# Autodesk Inventor assembly: CAR_011_VersaPlanetary_v2_Single_Stage_10_1_with_775_Series_Reverse
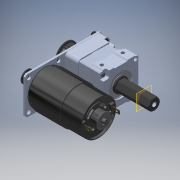
[picture p0: Inventor's stored thumbnail of the model, 180x180]
Saved by Autodesk Inventor 2018 (Build 220112000, 112)
## iProperties
Created: 2016-10-31
Part Number: CAR_011_VersaPlanetary_v2_Single_Stage_10_1_with_775_Series_Reverse
Description: STEP AP214
Document SubType Name: Assembly
Designer: Bobby's PC
Mass: 725.748 g
Surface Area: 818.615 cm^2
Volume: 178.451 cm^3
Density: 4.06694 g/cm^3
Sending System: SolidWorks 2016
Preprocessor: SwSTEP 2.0
Title: 217-4973_1stage_775pro.STEP
Revision Number: ANY
## Documents named in this file (16)
- C:\Users\user\Documents\GrabCAD\New folder\Build season\CAR_011_VersaPlanetary_v2_Single_Stage_10_1_with_775_Series_Reverse.iam
- C:\Users\user\Documents\GrabCAD\New folder\Build season\180 VERSAPLANETARY\217-2625-026 Rev1.ipt
- C:\Users\user\Documents\GrabCAD\New folder\Build season\180 VERSAPLANETARY\217-2742-001 Rev4.ipt
- C:\Users\user\Documents\GrabCAD\New folder\Build season\180 VERSAPLANETARY\217-2625-017 Rev1_9714K61.ipt
- C:\Users\user\Documents\GrabCAD\New folder\Build season\180 VERSAPLANETARY\217-2625-003 Rev1.ipt
- C:\Users\user\Documents\GrabCAD\New folder\Build season\180 VERSAPLANETARY\217-2625-018 Rev1_98541A410.ipt
- C:\Users\user\Documents\GrabCAD\New folder\Build season\180 VERSAPLANETARY\832-1750-Ring-Gear-Screw_SSA0832-0500ZC.ipt
- C:\Users\user\Documents\GrabCAD\New folder\Build season\180 VERSAPLANETARY\217-4649-002 Rev1_SSA0832-0500ZC.ipt
- C:\Users\user\Documents\GrabCAD\New folder\Build season\180 VERSAPLANETARY\217-4347-000 Rev1.ipt
- C:\Users\user\Documents\GrabCAD\New folder\Build season\180 VERSAPLANETARY\217-2820 Rev1_Public.iam
- C:\Users\user\Documents\GrabCAD\New folder\Build season\180 VERSAPLANETARY\217-2816-001 Rev1.ipt
- C:\Users\user\Documents\GrabCAD\New folder\Build season\180 VERSAPLANETARY\217-4649-007 Rev1_94105A824.ipt
- C:\Users\user\Documents\GrabCAD\New folder\Build season\180 VERSAPLANETARY\VersaPlanetary_180_Drive_-_Speed_Reducer.iam
- C:\Users\user\Documents\GrabCAD\New folder\Build season\180 VERSAPLANETARY\VersaPlanetary_180_Drive_Gusset_Kit.ipt
- C:\Users\user\Documents\GrabCAD\New folder\Build season\180 VERSAPLANETARY\12t_x_9mm_Wide_Double_Flange_Aluminum_Pulley_GT2_3mm_RS775_Motor_217-5871.ipt
- C:\Users\user\Documents\GrabCAD\New folder\Build season\180 VERSAPLANETARY\24t_x_9mm_Wide_Double_Flange_Aluminum_Pulley_GT2_3mm_1_2_Hex_Bore_217-5875.ipt
## Components (18 placed, 18 different names)
1. 217-2625-026 Rev1_1
2. 217-2742-001 Rev4_2
3. 217-2742-001 Rev4_3
4. 217-2625-017 Rev1_9714K61_4
5. 217-2625-003 Rev1_5
6. 217-2625-018 Rev1_98541A410_6
7. 832-1750-Ring-Gear-Screw_SSA0832-0500ZC_7 — Insert:10
8. 832-1750-Ring-Gear-Screw_SSA0832-0500ZC_8 — Mate:3, Mate:5
9. 217-4649-002 Rev1_SSA0832-0500ZC_10 — Insert:6
10. 217-4649-002 Rev1_SSA0832-0500ZC_11 — Insert:7, Mate:4
11. 217-4347-000 Rev1_15 — Mate:2, Insert:9, Mate:6
12. 217-2820 Rev1_Public_16 [sub-assembly]
13. 217-2816-001 Rev1_17 — Insert:3
14. 217-4649-007 Rev1_94105A824_19
15. VersaPlanetary_180_Drive_-_Speed_Reducer:1 [sub-assembly] — Insert:3, Insert:4, Insert:8, Mate:3, Mate:4, Mate:5
16. VersaPlanetary_180_Drive_Gusset_Kit:1 — Insert:4, Insert:6, Insert:7, Insert:9, Insert:10
17. 12t_x_9mm_Wide_Double_Flange_Aluminum_Pulley_GT2_3mm_RS775_Motor_217-5871:1 — Mate:2, Flush:2, Mate:6
18. 24t_x_9mm_Wide_Double_Flange_Aluminum_Pulley_GT2_3mm_1_2_Hex_Bore_217-5875:1 — Insert:8, Flush:2
## Relationships (13: Insert 7, Mate 5, Flush 1)
- Insert:3: 217-2816-001 Rev1_17 ↔ VersaPlanetary_180_Drive_-_Speed_Reducer:1
- Insert:4: VersaPlanetary_180_Drive_-_Speed_Reducer:1 ↔ VersaPlanetary_180_Drive_Gusset_Kit:1
- Insert:6 (3.175 mm): 217-4649-002 Rev1_SSA0832-0500ZC_10 ↔ VersaPlanetary_180_Drive_Gusset_Kit:1
- Insert:7: 217-4649-002 Rev1_SSA0832-0500ZC_11 ↔ VersaPlanetary_180_Drive_Gusset_Kit:1
- Insert:8: VersaPlanetary_180_Drive_-_Speed_Reducer:1 ↔ 24t_x_9mm_Wide_Double_Flange_Aluminum_Pulley_GT2_3mm_1_2_Hex_Bore_217-5875:1
- Mate:2: 217-4347-000 Rev1_15 ↔ 12t_x_9mm_Wide_Double_Flange_Aluminum_Pulley_GT2_3mm_RS775_Motor_217-5871:1
- Flush:2: 12t_x_9mm_Wide_Double_Flange_Aluminum_Pulley_GT2_3mm_RS775_Motor_217-5871:1 ↔ 24t_x_9mm_Wide_Double_Flange_Aluminum_Pulley_GT2_3mm_1_2_Hex_Bore_217-5875:1
- Mate:3: 832-1750-Ring-Gear-Screw_SSA0832-0500ZC_8 ↔ VersaPlanetary_180_Drive_-_Speed_Reducer:1
- Mate:4: 217-4649-002 Rev1_SSA0832-0500ZC_11 ↔ VersaPlanetary_180_Drive_-_Speed_Reducer:1
- Insert:9: 217-4347-000 Rev1_15 ↔ VersaPlanetary_180_Drive_Gusset_Kit:1
- Mate:5: 832-1750-Ring-Gear-Screw_SSA0832-0500ZC_8 ↔ VersaPlanetary_180_Drive_-_Speed_Reducer:1
- Mate:6: 217-4347-000 Rev1_15 ↔ 12t_x_9mm_Wide_Double_Flange_Aluminum_Pulley_GT2_3mm_RS775_Motor_217-5871:1
- Insert:10 (3.175 mm): 832-1750-Ring-Gear-Screw_SSA0832-0500ZC_7 ↔ VersaPlanetary_180_Drive_Gusset_Kit:1
